# Autodesk Inventor assembly: Assy_all
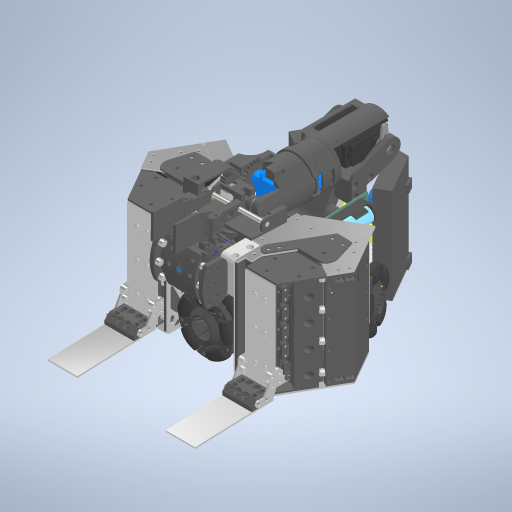
[picture p0: Inventor's stored thumbnail of the model, 512x512]
Saved by Autodesk Inventor 2024.1 (Build 281209000, 209)
## iProperties
Created: 2025-03-04
Part Number: Assy_all
Document SubType Name: Assembly
Designer: hibik
Author: hibik
## Documents named in this file (6)
- C:\Users\hibik\Documents\Robomech\RESCUE\ORCA\hard\Assy_all.iam
- C:\Users\hibik\Documents\Robomech\RESCUE\ORCA\hard\Assy_cam_connection.iam
- C:\Users\hibik\Documents\Robomech\RESCUE\ORCA\hard\flame_back\flame_back.ipt
- C:\Users\hibik\Documents\Robomech\RESCUE\ORCA\hard\board\core_power.iam
- C:\Users\hibik\Documents\Robomech\RESCUE\ORCA\hard\board\core_usp.iam
- C:\Users\hibik\Documents\Robomech\RESCUE\ORCA\hard\std_parts\battery.ipt
## Components (5 placed, 5 different names)
1. Assy_cam_connection:1 [sub-assembly] — メイト:1, フラッシュ:1, フラッシュ:2
2. flame_back:1 — メイト:1, フラッシュ:1, フラッシュ:2, 挿入:2, 挿入:3
3. core_power:1 [sub-assembly] — 挿入:2, 挿入:3
4. battery:1
5. core_usp:1 [sub-assembly]
## Relationships (5: Flush 2, Insert 2, Mate 1)
- メイト:1 [Mate]: Assy_cam_connection:1 ↔ flame_back:1
- フラッシュ:1 [Flush]: Assy_cam_connection:1 ↔ flame_back:1
- フラッシュ:2 [Flush]: Assy_cam_connection:1 ↔ flame_back:1
- 挿入:2 [Insert]: flame_back:1 ↔ core_power:1
- 挿入:3 [Insert]: flame_back:1 ↔ core_power:1
